# Autodesk Inventor assembly: Leg Long
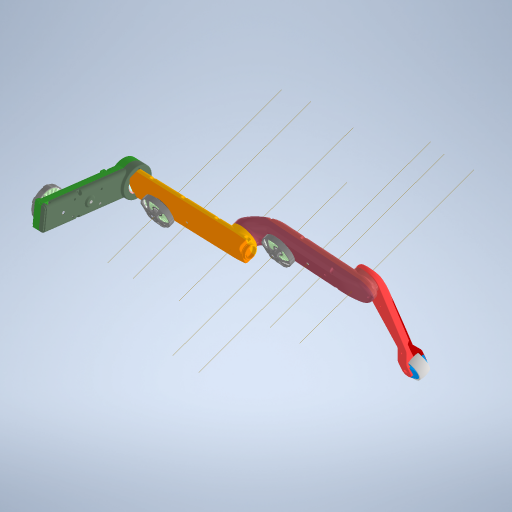
[picture p0: Inventor's stored thumbnail of the model, 512x512]
Saved by Autodesk Inventor 2023 (Build 270158000, 158)
## iProperties
Created: 2022-01-01
Part Number: Leg Long
Document SubType Name: Assembly
Designer: Jochen
Author: Jochen
## Documents named in this file (5)
- D:\Projects\Lisbeth\CAD\Leg Long.iam
- D:\Projects\Lisbeth\CAD\Thigh\Thigh.iam
- D:\Projects\Lisbeth\CAD\LowerLeg\LowerLeg.iam
- D:\Projects\Lisbeth\CAD\Lumbar\Lumbar Long.iam
- D:\Projects\Lisbeth\CAD\Hip\Hip Long.iam
## Components (4 placed, 4 different names)
1. Thigh:1 [sub-assembly] — Mate:6, Mate:7, Mate:10, Mate:11
2. LowerLeg:1 [sub-assembly] — Mate:6, Mate:7
3. Lumbar Long:1 [sub-assembly] — Mate:8, Mate:9
4. Hip:1 [sub-assembly] — Mate:8, Mate:9, Mate:10, Mate:11
## Relationships (6: Mate 6)
- Mate:6: Thigh:1 ↔ LowerLeg:1
- Mate:7: Thigh:1 ↔ LowerLeg:1
- Mate:8: Lumbar Long:1 ↔ Hip:1
- Mate:9: Lumbar Long:1 ↔ Hip:1
- Mate:10: Thigh:1 ↔ Hip:1
- Mate:11: Thigh:1 ↔ Hip:1
